# Autodesk Inventor assembly: ASY 700 water tray
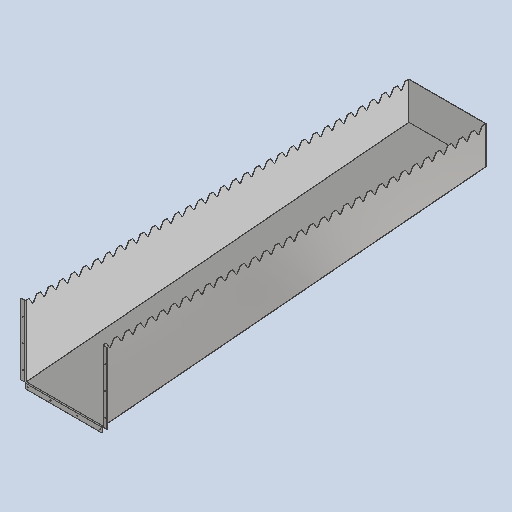
[picture p0: Inventor's stored thumbnail of the model, 512x512]
Saved by Autodesk Inventor 2025 (Build 290162010, 162A)
## iProperties
Created: 2024-09-09
Part Number: ASY 700 water tray
Document SubType Name: Assembly
Designer: user
Author: user
## Documents named in this file (5)
- C:\Users\DELL\YandexDisk-badmisterfox\домашниий пк\Inventor\Manturovo\Manturovo_Se-clar\ASY 700 water tray.iam
- C:\Users\DELL\YandexDisk-badmisterfox\домашниий пк\Inventor\Manturovo\Manturovo_Se-clar\MSC 706 ridge 1.ipt
- C:\Users\DELL\YandexDisk-badmisterfox\домашниий пк\Inventor\Manturovo\Manturovo_Se-clar\MSC 707 ridge 2.ipt
- C:\Users\DELL\YandexDisk-badmisterfox\домашниий пк\Inventor\Manturovo\Manturovo_Se-clar\MSC 708 ridge 4.ipt
- C:\Users\DELL\YandexDisk-badmisterfox\домашниий пк\Inventor\Manturovo\Manturovo_Se-clar\MSC 709 ridge 5.ipt
## Components (4 placed, 4 different names)
1. MSC 706 ridge 1:1
2. MSC 707 ridge 2:1
3. MSC 708 ridge 4:1
4. MSC 709 ridge 5:1
## Relationships (1: WeldJoint 1)
- [WeldJoint]: MSC 707 ridge 2:1 ↔ MSC 709 ridge 5:1
